# Autodesk Inventor assembly: 弹簧
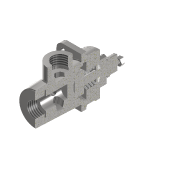
[picture p0: Inventor's stored thumbnail of the model, 180x180]
Saved by Autodesk Inventor 2022 (Build 260153000, 153)
## iProperties
Created: 2023-03-15
Part Number: 弹簧
Document SubType Name: Assembly
Designer: Lzy18
Author: Lzy18
## Documents named in this file (11)
- C:\Users\Lzy18\Desktop\20工2\弹簧.iam
- C:\Users\Lzy18\Desktop\20工2\阀体.ipt
- C:\Users\Lzy18\Desktop\20工2\旋塞.ipt
- C:\Users\Lzy18\Desktop\20工2\塞杆.ipt
- C:\Users\Lzy18\Desktop\20工2\螺盖.ipt
- C:\Users\Lzy18\Desktop\20工2\弹簧.ipt
- C:\Users\Lzy18\Desktop\20工2\垫片.ipt
- C:\Users\Lzy18\Desktop\20工2\胶垫.ipt
- C:\Users\Lzy18\Desktop\20工2\螺套.ipt
- C:\Users\Lzy18\Desktop\20工2\手柄.ipt
- C:\Users\Lzy18\Documents\Inventor\Content Center Files\R2022\zh-CN\GB_T 6170-2000\螺母 GB_T 6170 M12.ipt
## Components (10 placed, 10 different names)
1. 阀体:1 — 配合:1, 配合:13, 表面齐平:3
2. 旋塞:1 — 配合:1, 配合:2, 配合:3, 表面齐平:2
3. 塞杆:1 — 配合:2, 配合:3, 配合:4, 配合:5, 配合:10, 配合:11, 插入:2
4. 螺盖:1 — 配合:4, 配合:5, 表面齐平:1, 配合:6, 配合:7, 配合:8, 配合:9, 配合:13
5. 弹簧:1 — 表面齐平:1
6. 垫片:1 — 配合:6, 配合:7
7. 胶垫:2 — 配合:8, 配合:9, 插入:1
8. 螺套:1 — 插入:1, 配合:12
9. 手柄:1 — 配合:10, 配合:11, 配合:12
10. 螺母 GB/T 6170-2000 M12:1 — 插入:2
## Relationships (19: Mate 13, Flush 4, Insert 2)
- 配合:1 [Mate]: 阀体:1 ↔ 旋塞:1
- 配合:2 [Mate]: 旋塞:1 ↔ 塞杆:1
- 配合:3 [Mate]: 旋塞:1 ↔ 塞杆:1
- 配合:4 [Mate]: 塞杆:1 ↔ 螺盖:1
- 配合:5 [Mate] (33.5 mm): 塞杆:1 ↔ 螺盖:1
- 表面齐平:1 [Flush]: 螺盖:1 ↔ 弹簧:1
- 配合:6 [Mate]: 螺盖:1 ↔ 垫片:1
- 配合:7 [Mate] (1 mm): 螺盖:1 ↔ 垫片:1
- 配合:8 [Mate]: 螺盖:1 ↔ 胶垫:2
- 配合:9 [Mate]: 螺盖:1 ↔ 胶垫:2
- 插入:1 [Insert]: 胶垫:2 ↔ 螺套:1
- 配合:10 [Mate]: 塞杆:1 ↔ 手柄:1
- 配合:11 [Mate]: 塞杆:1 ↔ 手柄:1
- 配合:12 [Mate]: 螺套:1 ↔ 手柄:1
- 插入:2 [Insert]: 塞杆:1 ↔ 螺母 GB/T 6170-2000 M12:1
- 配合:13 [Mate] (3.216 mm): 阀体:1 ↔ 螺盖:1
- 表面齐平:2 [Flush] (-39.28 mm): 旋塞:1
- 表面齐平:3 [Flush] (-70 mm): 阀体:1
- 表面齐平:4 [Flush]
